# Autodesk Inventor assembly: BodyBot
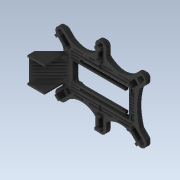
[picture p0: Inventor's stored thumbnail of the model, 180x180]
Saved by Autodesk Inventor 2020 (Build 240168000, 168)
## iProperties
Created: 2021-03-17
Part Number: BodyBot
Document SubType Name: Assembly
Designer: Turing
Author: Turing
## Documents named in this file (3)
- D:\Hexapod3DPrint\BodyBot.iam
- D:\Hexapod3DPrint\BodyBot2.ipt
- D:\Hexapod3DPrint\BodyBot1.ipt
## Components (2 placed, 2 different names)
1. BodyBot2:1 — Rigid:1
2. BodyBot1:1 — Rigid:1
## Relationships (1: WeldJoint 1)
- Rigid:1 [WeldJoint]: BodyBot2:1 ↔ BodyBot1:1
